# Autodesk Inventor assembly: assembily_v2
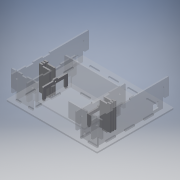
[picture p0: Inventor's stored thumbnail of the model, 180x180]
Saved by Autodesk Inventor 2017.2 (Build 212233000, 233)
## iProperties
Created: 2017-06-09
Part Number: assembily_v2
Document SubType Name: Assembly
Designer: SandeepSH
Author: SandeepSH
## Documents named in this file (13)
- C:\Users\SandeepSH\Dropbox\MSC\Project\inventor\lcv1\assembily_v2.iam
- C:\Users\SandeepSH\Dropbox\MSC\Project\inventor\lcv1\base_v2.ipt
- C:\Users\SandeepSH\Dropbox\MSC\Project\inventor\lcv1\cham_right_v2.ipt
- C:\Users\SandeepSH\Dropbox\MSC\Project\inventor\lcv1\cham_left_v2.ipt
- C:\Users\SandeepSH\Dropbox\MSC\Project\inventor\lcv1\cham_back_v2.ipt
- C:\Users\SandeepSH\Dropbox\MSC\Project\inventor\lcv1\front_left_v2.ipt
- C:\Users\SandeepSH\Dropbox\MSC\Project\inventor\lcv1\front_right_v2.ipt
- C:\Users\SandeepSH\Dropbox\MSC\Project\inventor\lcv1\hollow_mount.ipt
- C:\Users\SandeepSH\Dropbox\MSC\Project\inventor\lcv1\fill_mount.ipt
- C:\Users\SandeepSH\Dropbox\MSC\Project\inventor\lcv1\side_v2.ipt
- C:\Users\SandeepSH\Dropbox\MSC\Project\inventor\lcv1\top_right_v2.ipt
- C:\Users\SandeepSH\Dropbox\MSC\Project\inventor\lcv1\roof_v2.ipt
- C:\Users\SandeepSH\Dropbox\MSC\Project\inventor\lcv1\hangar.ipt
## Components (18 placed, 12 different names)
1. base_v2:1 — Mate:5, Mate:6, Mate:7, Mate:8, Mate:9, Mate:10, Mate:11, Mate:12, Mate:13, Mate:14, Mate:15, Mate:16, Mate:17, Mate:18, Mate:19, Mate:20, Mate:21, Mate:22, Mate:23, Mate:24, Mate:25, Mate:26, Mate:27, Mate:28, Mate:29
2. cham_back_v2:1 — Mate:5, Mate:6
3. cham_left_v2:1 — Mate:7
4. cham_right_v2:1 — Mate:8, Mate:9
5. front_right_v2:1 — Mate:10, Mate:11, Mate:30, Mate:31
6. front_left_v2:1 — Mate:12, Mate:13
7. hollow_mount:1 — Mate:14, Mate:15
8. hollow_mount:2 — Mate:16, Mate:17
9. fill_mount:1 — Mate:18, Mate:19
10. fill_mount:2 — Mate:20, Mate:21
11. fill_mount:3 — Mate:22, Mate:23
12. fill_mount:4 — Mate:24, Mate:25
13. side_v2:1 — Mate:26, Mate:27
14. side_v2:2 — Mate:28, Mate:29
15. top_right_v2:1 — Mate:30, Mate:31
16. roof_v2:1 — Mate:32, Mate:33, Mate:34, Mate:35, Mate:36
17. hangar:1 — Mate:32, Mate:33, Mate:34
18. hangar:2 — Mate:35, Mate:36
## Relationships (32: Mate 32)
- Mate:5: base_v2:1 ↔ cham_back_v2:1
- Mate:6: base_v2:1 ↔ cham_back_v2:1
- Mate:7: base_v2:1 ↔ cham_left_v2:1
- Mate:8: base_v2:1 ↔ cham_right_v2:1
- Mate:9: base_v2:1 ↔ cham_right_v2:1
- Mate:10: base_v2:1 ↔ front_right_v2:1
- Mate:11: base_v2:1 ↔ front_right_v2:1
- Mate:12: base_v2:1 ↔ front_left_v2:1
- Mate:13: base_v2:1 ↔ front_left_v2:1
- Mate:14: base_v2:1 ↔ hollow_mount:1
- Mate:15: base_v2:1 ↔ hollow_mount:1
- Mate:16: base_v2:1 ↔ hollow_mount:2
- Mate:17: base_v2:1 ↔ hollow_mount:2
- Mate:18: base_v2:1 ↔ fill_mount:1
- Mate:19: base_v2:1 ↔ fill_mount:1
- Mate:20: base_v2:1 ↔ fill_mount:2
- Mate:21: base_v2:1 ↔ fill_mount:2
- Mate:22: base_v2:1 ↔ fill_mount:3
- Mate:23: base_v2:1 ↔ fill_mount:3
- Mate:24: base_v2:1 ↔ fill_mount:4
- Mate:25: base_v2:1 ↔ fill_mount:4
- Mate:26: base_v2:1 ↔ side_v2:1
- Mate:27: base_v2:1 ↔ side_v2:1
- Mate:28: base_v2:1 ↔ side_v2:2
- Mate:29: base_v2:1 ↔ side_v2:2
- Mate:30: front_right_v2:1 ↔ top_right_v2:1
- Mate:31: front_right_v2:1 ↔ top_right_v2:1
- Mate:32: roof_v2:1 ↔ hangar:1
- Mate:33: roof_v2:1 ↔ hangar:1
- Mate:34: roof_v2:1 ↔ hangar:1
- Mate:35: roof_v2:1 ↔ hangar:2
- Mate:36: roof_v2:1 ↔ hangar:2
